# Autodesk Inventor assembly: Shoulder base
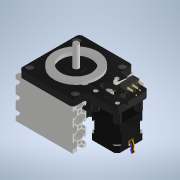
[picture p0: Inventor's stored thumbnail of the model, 180x180]
Saved by Autodesk Inventor 2022 (Build 260153000, 153)
## iProperties
Created: 2022-03-02
Part Number: Shoulder base
Document SubType Name: Assembly
Designer: JK
Author: JK
## Documents named in this file (24)
- C:\Users\JK\Documents\Inventor\ScaraNema\SCARA-3DP\Parts\Shoulder\Shoulder base.iam
- C:\Users\JK\Documents\Inventor\ScaraNema\SCARA-3DP\Parts\Shoulder\Needle roller bearing\5909K79_1 mm Thick Washer for 45 mm Shaft Diameter Needle-Roller Thrust Bearing.ipt
- C:\Users\JK\Documents\Inventor\ScaraNema\SCARA-3DP\Parts\Shoulder\Needle roller bearing\5909K19_Needle-Roller Thrust Bearing.ipt
- C:\Users\JK\Documents\Inventor\ScaraNema\SCARA-3DP\Parts\Common components\GT2 16 Pulley.ipt
- C:\Users\JK\Documents\Inventor\ScaraNema\SCARA-3DP\Parts\Arm\8x80 mm axis.ipt
- C:\Users\JK\Documents\Inventor\ScaraNema\SCARA-3DP\Parts\Common components\GT260T.ipt
- C:\Users\JK\Documents\Inventor\ScaraNema\SCARA-3DP\Parts\Common components\Motor.ipt
- C:\Users\JK\Documents\Inventor\ScaraNema\SCARA-3DP\Parts\Shoulder\Shoulder top base.ipt
- C:\Users\JK\Documents\Inventor\ScaraNema\SCARA-3DP\Parts\Shoulder\V-Slot 20x60x85.ipt
- C:\Users\JK\Documents\Inventor\ScaraNema\SCARA-3DP\Parts\Shoulder\Shoulder bottom base.ipt
- C:\Users\JK\Documents\Inventor\ScaraNema\SCARA-3DP\Parts\Shoulder\shoulder motor separator.ipt
- C:\Users\JK\Documents\Inventor\ScaraNema\SCARA-3DP\Parts\Fasteners\M5 Hex nut.ipt
- C:\Users\JK\Documents\Inventor\ScaraNema\SCARA-3DP\Parts\Shoulder\Shoulder base separator.ipt
- C:\Users\JK\Documents\Inventor\ScaraNema\SCARA-3DP\Parts\Shoulder\Arm limit switch support.ipt
- C:\Users\JK\Documents\Inventor\ScaraNema\SCARA-3DP\Parts\Common components\Limit switch.ipt
- C:\Users\JK\Documents\Inventor\ScaraNema\SCARA-3DP\Parts\Fasteners\M3x25 socket solt.ipt
- C:\Users\JK\Documents\Inventor\ScaraNema\SCARA-3DP\Parts\Fasteners\M3 Hex nut.ipt
- C:\Users\JK\Documents\Inventor\ScaraNema\SCARA-3DP\Parts\Fasteners\M5x12 Flat head bolt.ipt
- C:\Users\JK\Documents\Inventor\ScaraNema\SCARA-3DP\Parts\Fasteners\M5x45 Flat head bolt.ipt
- C:\Users\JK\Documents\Inventor\ScaraNema\SCARA-3DP\Parts\Fasteners\M5 T-Nut Drop-in 20x20.ipt
- C:\Users\JK\Documents\Inventor\ScaraNema\SCARA-3DP\Parts\Fasteners\M3x15 socket bolt.ipt
- C:\Users\JK\Documents\Inventor\ScaraNema\SCARA-3DP\Parts\Fasteners\M2 Hex nut.ipt
- C:\Users\JK\Documents\Inventor\ScaraNema\SCARA-3DP\Parts\Fasteners\M2x10 socket bolt.ipt
- C:\Users\JK\Documents\Inventor\ScaraNema\SCARA-3DP\Parts\Common components\688-2RS.ipt
## Components (59 placed, 23 different names)
1. 5909K79_1 mm Thick Washer for 45 mm Shaft Diameter Needle-Roller Thrust Bearing:1 — Tangente:1, Coincidencia:45, Coincidencia:51
2. 5909K19_Needle-Roller Thrust Bearing:1 — Tangente:1, Tangente:2, Coincidencia:45, Coincidencia:46
3. 5909K79_1 mm Thick Washer for 45 mm Shaft Diameter Needle-Roller Thrust Bearing:2 — Tangente:2, Coincidencia:148
4. 8x80 mm axis:1 — Coincidencia:41, Coincidencia:46, Coincidencia:50, Coincidencia:144, Coincidencia:145, Nivelación:42, Coincidencia:148
5. GT260T:1 — Coincidencia:41, Coincidencia:60, Coincidencia:62, Nivelación:17
6. Motor:1 — Ángulo:4, Coincidencia:67, Coincidencia:68, Coincidencia:70
7. GT2 16 Pulley:2 — Coincidencia:67, Nivelación:17, Coincidencia:68, Coincidencia:72
8. Shoulder top base:1 — Coincidencia:50, Coincidencia:51, Ángulo:3, Ángulo:4, Coincidencia:57, Coincidencia:58, Nivelación:13, Nivelación:14, Nivelación:16, Coincidencia:62, Coincidencia:71, Coincidencia:72, Coincidencia:75, Coincidencia:78, Ángulo:7, Nivelación:20, Coincidencia:82, Ángulo:8, Coincidencia:91, Coincidencia:92, Coincidencia:93, Coincidencia:94, Coincidencia:95, Coincidencia:102, Coincidencia:103, Coincidencia:105, Coincidencia:109, Coincidencia:119, Coincidencia:120, Ángulo:14, Coincidencia:121, Coincidencia:122, Coincidencia:123, Coincidencia:146
9. V-Slot 20x60x85:1 — Coincidencia:57, Nivelación:14, Nivelación:15, Nivelación:19, Ángulo:5, Ángulo:12
10. V-Slot 20x60x85:2 — Coincidencia:58, Nivelación:13, Nivelación:15, Nivelación:16
11. Shoulder bottom base:1 — Coincidencia:60, Nivelación:18, Nivelación:19, Ángulo:5, Coincidencia:83, Coincidencia:84, Ángulo:9, Coincidencia:96, Coincidencia:97, Coincidencia:98, Coincidencia:99, Coincidencia:100, Coincidencia:101, Coincidencia:114, Coincidencia:117, Coincidencia:147, Nivelación:42
12. Arm limit switch support:1 — Coincidencia:78, Coincidencia:80, Coincidencia:81, Ángulo:6, Ángulo:7, Nivelación:20, Coincidencia:82, Ángulo:8, Coincidencia:124, Ángulo:20, Coincidencia:140
13. Limit switch:1 — Coincidencia:80, Coincidencia:81, Ángulo:6, Coincidencia:138, Coincidencia:139, Coincidencia:141, Coincidencia:142, Coincidencia:143
14. M5x12 Flat head bolt:1 — Coincidencia:92, Nivelación:24, Nivelación:25, Coincidencia:95, Coincidencia:111
15. M5x12 Flat head bolt:2 — Coincidencia:93, Nivelación:25, Coincidencia:112
16. M5x12 Flat head bolt:3 — Coincidencia:91, Nivelación:23, Nivelación:24, Coincidencia:110
17. M5x12 Flat head bolt:4 — Coincidencia:94, Nivelación:23, Coincidencia:108
18. M5x12 Flat head bolt:5 — Coincidencia:96, Nivelación:27, Coincidencia:100, Coincidencia:115
19. M5x12 Flat head bolt:6 — Coincidencia:99, Nivelación:26, Coincidencia:118
20. M5x12 Flat head bolt:7 — Coincidencia:98, Nivelación:26, Coincidencia:101, Coincidencia:116
21. M5x12 Flat head bolt:8 — Coincidencia:97, Nivelación:27, Coincidencia:113
22. M5 T-Nut Drop-in 20x20:2 — Nivelación:28, Nivelación:29, Nivelación:30, Coincidencia:111
23. M5 T-Nut Drop-in 20x20:3 — Nivelación:30, Coincidencia:110
24. M5 T-Nut Drop-in 20x20:4 — Nivelación:29, Coincidencia:112
25. M5 T-Nut Drop-in 20x20:1 — Coincidencia:108, Coincidencia:109, Ángulo:12, Nivelación:28
26. M5 T-Nut Drop-in 20x20:5 — Coincidencia:118, Nivelación:32
27. M5 T-Nut Drop-in 20x20:6 — Coincidencia:116, Coincidencia:117, Nivelación:32
28. M5 T-Nut Drop-in 20x20:7 — Nivelación:31, Coincidencia:115
29. M5 T-Nut Drop-in 20x20:8 — Coincidencia:113, Coincidencia:114, Nivelación:31
30. M3 Hex nut:3 — Coincidencia:119, Nivelación:33, Ángulo:13
31. M3 Hex nut:4 — Coincidencia:120, Nivelación:33, Ángulo:13, Ángulo:14, Coincidencia:121
32. M3x15 socket bolt:1 — Coincidencia:122, Nivelación:34, Coincidencia:124
33. M3x15 socket bolt:2 — Coincidencia:123, Nivelación:34
34. M2 Hex nut:1 — Coincidencia:138, Ángulo:19, Ángulo:20, Nivelación:40, Coincidencia:140
35. M2 Hex nut:2 — Coincidencia:139, Ángulo:19, Nivelación:40
36. M2x10 socket bolt:1 — Coincidencia:141, Nivelación:41, Coincidencia:143
37. M2x10 socket bolt:2 — Coincidencia:142, Nivelación:41
38. 688-2RS:1 — Coincidencia:144, Coincidencia:147
39. 688-2RS:2 — Coincidencia:145, Coincidencia:146
40. shoulder motor separator:1 — Coincidencia:70, Coincidencia:71, Coincidencia:104
41. shoulder motor separator:2
42. shoulder motor separator:3
43. shoulder motor separator:4
44. Shoulder base separator:1 — Coincidencia:75, Coincidencia:83
45. Shoulder base separator:2
46. Shoulder base separator:3
47. Shoulder base separator:4
48. M5 Hex nut:2 — Nivelación:18, Coincidencia:84, Ángulo:9
49. M5 Hex nut:3
50. M5 Hex nut:4
51. M5 Hex nut:5
52. M5x45 Flat head bolt:1 — Coincidencia:102, Coincidencia:103
53. M5x45 Flat head bolt:2
54. M5x45 Flat head bolt:3
55. M5x45 Flat head bolt:4
56. M3x25 socket solt:3 — Coincidencia:104, Coincidencia:105
57. M3x25 socket solt:4
58. M3x25 socket solt:5
59. M3x25 socket solt:6
## Component patterns: (4 elements, first: shoulder motor separator:1), (4 elements, first: Shoulder base separator:1), (4 elements, first: M5 Hex nut:2), (4 elements, first: M5x45 Flat head bolt:1), (4 elements, first: M3x25 socket solt:3)
## Relationships (101: Mate 64, Flush 23, Angle 12, Tangent 2)
- Tangente:1: 5909K79_1 mm Thick Washer for 45 mm Shaft Diameter Needle-Roller Thrust Bearing:1 ↔ 5909K19_Needle-Roller Thrust Bearing:1
- Tangente:2: 5909K19_Needle-Roller Thrust Bearing:1 ↔ 5909K79_1 mm Thick Washer for 45 mm Shaft Diameter Needle-Roller Thrust Bearing:2
- Coincidencia:41 [Mate]: 8x80 mm axis:1 ↔ GT260T:1
- Coincidencia:45 [Mate]: 5909K79_1 mm Thick Washer for 45 mm Shaft Diameter Needle-Roller Thrust Bearing:1 ↔ 5909K19_Needle-Roller Thrust Bearing:1
- Coincidencia:46 [Mate]: 5909K19_Needle-Roller Thrust Bearing:1 ↔ 8x80 mm axis:1
- Coincidencia:50 [Mate]: 8x80 mm axis:1 ↔ Shoulder top base:1
- Coincidencia:51 [Mate]: 5909K79_1 mm Thick Washer for 45 mm Shaft Diameter Needle-Roller Thrust Bearing:1 ↔ Shoulder top base:1
- Ángulo:3 [Angle] (0 deg): Shoulder top base:1
- Ángulo:4 [Angle] (0 deg): Motor:1 ↔ Shoulder top base:1
- Coincidencia:57 [Mate]: Shoulder top base:1 ↔ V-Slot 20x60x85:1
- Coincidencia:58 [Mate]: Shoulder top base:1 ↔ V-Slot 20x60x85:2
- Nivelación:13 [Flush]: Shoulder top base:1 ↔ V-Slot 20x60x85:2
- Nivelación:14 [Flush]: Shoulder top base:1 ↔ V-Slot 20x60x85:1
- Nivelación:15 [Flush]: V-Slot 20x60x85:1 ↔ V-Slot 20x60x85:2
- Nivelación:16 [Flush]: Shoulder top base:1 ↔ V-Slot 20x60x85:2
- Coincidencia:60 [Mate]: GT260T:1 ↔ Shoulder bottom base:1
- Coincidencia:62 [Mate] (1 mm): GT260T:1 ↔ Shoulder top base:1
- Coincidencia:67 [Mate] (3 mm): Motor:1 ↔ GT2 16 Pulley:2
- Nivelación:17 [Flush]: GT260T:1 ↔ GT2 16 Pulley:2
- Coincidencia:68 [Mate]: Motor:1 ↔ GT2 16 Pulley:2
- Coincidencia:70 [Mate]: Motor:1 ↔ shoulder motor separator:1
- Coincidencia:71 [Mate]: Shoulder top base:1 ↔ shoulder motor separator:1
- Coincidencia:72 [Mate]: GT2 16 Pulley:2 ↔ Shoulder top base:1
- Nivelación:18 [Flush]: Shoulder bottom base:1 ↔ M5 Hex nut:2
- Coincidencia:75 [Mate]: Shoulder top base:1 ↔ Shoulder base separator:1
- Nivelación:19 [Flush] (21 mm): V-Slot 20x60x85:1 ↔ Shoulder bottom base:1
- Ángulo:5 [Angle] (0 deg): V-Slot 20x60x85:1 ↔ Shoulder bottom base:1
- Coincidencia:78 [Mate]: Shoulder top base:1 ↔ Arm limit switch support:1
- Coincidencia:80 [Mate]: Arm limit switch support:1 ↔ Limit switch:1
- Coincidencia:81 [Mate]: Arm limit switch support:1 ↔ Limit switch:1
- Ángulo:6 [Angle] (0 deg): Arm limit switch support:1 ↔ Limit switch:1
- Ángulo:7 [Angle] (0 deg): Shoulder top base:1 ↔ Arm limit switch support:1
- Nivelación:20 [Flush] (12.5 mm): Shoulder top base:1 ↔ Arm limit switch support:1
- Coincidencia:82 [Mate]: Shoulder top base:1 ↔ Arm limit switch support:1
- Ángulo:8 [Angle] (0 deg): Shoulder top base:1 ↔ Arm limit switch support:1
- Coincidencia:83 [Mate]: Shoulder bottom base:1 ↔ Shoulder base separator:1
- Coincidencia:84 [Mate]: Shoulder bottom base:1 ↔ M5 Hex nut:2
- Ángulo:9 [Angle] (0 deg): Shoulder bottom base:1 ↔ M5 Hex nut:2
- Coincidencia:91 [Mate]: Shoulder top base:1 ↔ M5x12 Flat head bolt:3
- Coincidencia:92 [Mate]: Shoulder top base:1 ↔ M5x12 Flat head bolt:1
- Coincidencia:93 [Mate]: Shoulder top base:1 ↔ M5x12 Flat head bolt:2
- Coincidencia:94 [Mate]: Shoulder top base:1 ↔ M5x12 Flat head bolt:4
- Nivelación:23 [Flush]: M5x12 Flat head bolt:3 ↔ M5x12 Flat head bolt:4
- Nivelación:24 [Flush]: M5x12 Flat head bolt:1 ↔ M5x12 Flat head bolt:3
- Nivelación:25 [Flush]: M5x12 Flat head bolt:1 ↔ M5x12 Flat head bolt:2
- Coincidencia:95 [Mate]: Shoulder top base:1 ↔ M5x12 Flat head bolt:1
- Coincidencia:96 [Mate]: Shoulder bottom base:1 ↔ M5x12 Flat head bolt:5
- Coincidencia:97 [Mate]: Shoulder bottom base:1 ↔ M5x12 Flat head bolt:8
- Coincidencia:98 [Mate]: Shoulder bottom base:1 ↔ M5x12 Flat head bolt:7
- Coincidencia:99 [Mate]: Shoulder bottom base:1 ↔ M5x12 Flat head bolt:6
- Nivelación:26 [Flush]: M5x12 Flat head bolt:6 ↔ M5x12 Flat head bolt:7
- Nivelación:27 [Flush]: M5x12 Flat head bolt:5 ↔ M5x12 Flat head bolt:8
- Coincidencia:100 [Mate]: Shoulder bottom base:1 ↔ M5x12 Flat head bolt:5
- Coincidencia:101 [Mate]: Shoulder bottom base:1 ↔ M5x12 Flat head bolt:7
- Coincidencia:102 [Mate]: Shoulder top base:1 ↔ M5x45 Flat head bolt:1
- Coincidencia:103 [Mate]: Shoulder top base:1 ↔ M5x45 Flat head bolt:1
- Coincidencia:104 [Mate]: shoulder motor separator:1 ↔ M3x25 socket solt:3
- Coincidencia:105 [Mate]: Shoulder top base:1 ↔ M3x25 socket solt:3
- Coincidencia:108 [Mate]: M5x12 Flat head bolt:4 ↔ M5 T-Nut Drop-in 20x20:1
- Coincidencia:109 [Mate] (0.6 mm): Shoulder top base:1 ↔ M5 T-Nut Drop-in 20x20:1
- Ángulo:12 [Angle] (0 deg): V-Slot 20x60x85:1 ↔ M5 T-Nut Drop-in 20x20:1
- Nivelación:28 [Flush]: M5 T-Nut Drop-in 20x20:2 ↔ M5 T-Nut Drop-in 20x20:1
- Nivelación:29 [Flush]: M5 T-Nut Drop-in 20x20:2 ↔ M5 T-Nut Drop-in 20x20:4
- Nivelación:30 [Flush]: M5 T-Nut Drop-in 20x20:2 ↔ M5 T-Nut Drop-in 20x20:3
- Coincidencia:110 [Mate]: M5x12 Flat head bolt:3 ↔ M5 T-Nut Drop-in 20x20:3
- Coincidencia:111 [Mate]: M5x12 Flat head bolt:1 ↔ M5 T-Nut Drop-in 20x20:2
- Coincidencia:112 [Mate]: M5x12 Flat head bolt:2 ↔ M5 T-Nut Drop-in 20x20:4
- Coincidencia:113 [Mate]: M5x12 Flat head bolt:8 ↔ M5 T-Nut Drop-in 20x20:8
- Coincidencia:114 [Mate] (0.6 mm): Shoulder bottom base:1 ↔ M5 T-Nut Drop-in 20x20:8
- Nivelación:31 [Flush]: M5 T-Nut Drop-in 20x20:7 ↔ M5 T-Nut Drop-in 20x20:8
- Coincidencia:115 [Mate]: M5x12 Flat head bolt:5 ↔ M5 T-Nut Drop-in 20x20:7
- Coincidencia:116 [Mate]: M5x12 Flat head bolt:7 ↔ M5 T-Nut Drop-in 20x20:6
- Coincidencia:117 [Mate] (0.6 mm): Shoulder bottom base:1 ↔ M5 T-Nut Drop-in 20x20:6
- Coincidencia:118 [Mate]: M5x12 Flat head bolt:6 ↔ M5 T-Nut Drop-in 20x20:5
- Nivelación:32 [Flush]: M5 T-Nut Drop-in 20x20:5 ↔ M5 T-Nut Drop-in 20x20:6
- Coincidencia:119 [Mate]: Shoulder top base:1 ↔ M3 Hex nut:3
- Coincidencia:120 [Mate]: Shoulder top base:1 ↔ M3 Hex nut:4
- Nivelación:33 [Flush]: M3 Hex nut:3 ↔ M3 Hex nut:4
- Ángulo:13 [Angle] (0 deg): M3 Hex nut:3 ↔ M3 Hex nut:4
- Ángulo:14 [Angle] (0 deg): Shoulder top base:1 ↔ M3 Hex nut:4
- Coincidencia:121 [Mate]: Shoulder top base:1 ↔ M3 Hex nut:4
- Coincidencia:122 [Mate]: Shoulder top base:1 ↔ M3x15 socket bolt:1
- Coincidencia:123 [Mate]: Shoulder top base:1 ↔ M3x15 socket bolt:2
- Nivelación:34 [Flush]: M3x15 socket bolt:1 ↔ M3x15 socket bolt:2
- Coincidencia:124 [Mate]: Arm limit switch support:1 ↔ M3x15 socket bolt:1
- Coincidencia:138 [Mate]: Limit switch:1 ↔ M2 Hex nut:1
- Coincidencia:139 [Mate]: Limit switch:1 ↔ M2 Hex nut:2
- Ángulo:19 [Angle] (0 deg): M2 Hex nut:1 ↔ M2 Hex nut:2
- Ángulo:20 [Angle] (0 deg): Arm limit switch support:1 ↔ M2 Hex nut:1
- Nivelación:40 [Flush]: M2 Hex nut:1 ↔ M2 Hex nut:2
- Coincidencia:140 [Mate]: Arm limit switch support:1 ↔ M2 Hex nut:1
- Coincidencia:141 [Mate]: Limit switch:1 ↔ M2x10 socket bolt:1
- Coincidencia:142 [Mate]: Limit switch:1 ↔ M2x10 socket bolt:2
- Nivelación:41 [Flush]: M2x10 socket bolt:1 ↔ M2x10 socket bolt:2
- Coincidencia:143 [Mate]: Limit switch:1 ↔ M2x10 socket bolt:1
- Coincidencia:144 [Mate]: 8x80 mm axis:1 ↔ 688-2RS:1
- Coincidencia:145 [Mate]: 8x80 mm axis:1 ↔ 688-2RS:2
- Coincidencia:146 [Mate]: Shoulder top base:1 ↔ 688-2RS:2
- Coincidencia:147 [Mate]: Shoulder bottom base:1 ↔ 688-2RS:1
- Nivelación:42 [Flush]: 8x80 mm axis:1 ↔ Shoulder bottom base:1
- Coincidencia:148 [Mate]: 5909K79_1 mm Thick Washer for 45 mm Shaft Diameter Needle-Roller Thrust Bearing:2 ↔ 8x80 mm axis:1
